# Autodesk Inventor assembly: zlozenie_blotnik_v3
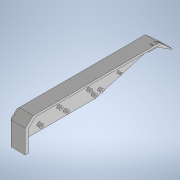
[picture p0: Inventor's stored thumbnail of the model, 180x180]
Saved by Autodesk Inventor 2022.3 (Build 263350000, 350)
## iProperties
Created: 2022-10-27
Part Number: zlozenie_blotnik_v3
Document SubType Name: Assembly
Designer: komputer
Author: komputer
## Documents named in this file (4)
- C:\Users\komputer\Desktop\zlozenie_blotnik_v3.iam
- C:\Users\komputer\Desktop\błotnik_v2.ipt
- C:\Users\komputer\zaślepka-1.ipt
- C:\Users\komputer\zaslepka_sruby-1.ipt
## Components (3 placed, 3 different names)
1. błotnik_v2:1 — Flush:1, Flush:2, Flush:3, Flush:4, Flush:5
2. zaślepka-1:1 — Flush:1, Flush:2, Flush:3
3. zaslepka_sruby-1:1 — Flush:4, Flush:5
## Relationships (5: Flush 5)
- Flush:1: błotnik_v2:1 ↔ zaślepka-1:1
- Flush:2: błotnik_v2:1 ↔ zaślepka-1:1
- Flush:3: błotnik_v2:1 ↔ zaślepka-1:1
- Flush:4: błotnik_v2:1 ↔ zaslepka_sruby-1:1
- Flush:5: błotnik_v2:1 ↔ zaslepka_sruby-1:1
